# Autodesk Inventor assembly: Cam Follower - Complete
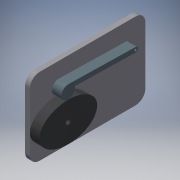
[picture p0: Inventor's stored thumbnail of the model, 180x180]
Saved by Autodesk Inventor 2016 (Build 200138000, 138)
## iProperties
Created: 2014-03-13
Part Number: Cam Follower - Complete
Document SubType Name: Assembly
Designer: John
Author: John
## Documents named in this file (4)
- C:\File Storage\Autodesk\Inventor 2016 Projects\Ex_Files_Inventor_2016_EssT\Exercise Files\15_Using constraints to position parts\15_05\Cam Follower - Complete.iam
- C:\File Storage\Autodesk\Inventor 2016 Projects\Ex_Files_Inventor_2016_EssT\Exercise Files\15_Using constraints to position parts\15_05\Base.ipt
- C:\File Storage\Autodesk\Inventor 2016 Projects\Ex_Files_Inventor_2016_EssT\Exercise Files\15_Using constraints to position parts\15_05\Arm.ipt
- C:\File Storage\Autodesk\Inventor 2016 Projects\Ex_Files_Inventor_2016_EssT\Exercise Files\15_Using constraints to position parts\15_05\Cam.ipt
## Components (3 placed, 3 different names)
1. Base:1 — Mate:1, Mate:2, Mate:3, Mate:4, Angle:1
2. Arm:1 — Mate:1, Mate:2, Transitional:1
3. Cam:1 — Mate:3, Mate:4, Angle:1, Transitional:1
## Relationships (6: Mate 4, Angle 1, Transitional 1)
- Mate:1: Base:1 ↔ Arm:1
- Mate:2: Base:1 ↔ Arm:1
- Mate:3: Base:1 ↔ Cam:1
- Mate:4: Base:1 ↔ Cam:1
- Angle:1 (0 deg): Base:1 ↔ Cam:1
- Transitional:1: Arm:1 ↔ Cam:1
